# Autodesk Inventor assembly: motormount_new
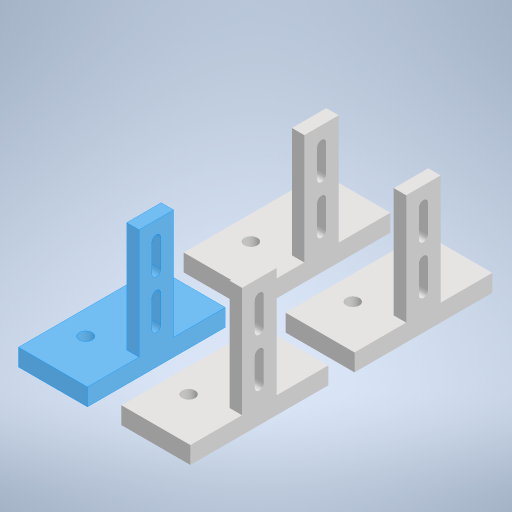
[picture p0: Inventor's stored thumbnail of the model, 512x512]
Saved by Autodesk Inventor 2024 (Build 280153000, 153)
## iProperties
Created: 2023-12-05
Part Number: motormount_new
Document SubType Name: Assembly
Designer: dimademler
Author: dimademler
## Documents named in this file (2)
- \\Mac\Home\Desktop\UCSD\2023-2024\Quarter_1\Physics_124\CAD new motor\motormount_new.iam
- \\Mac\Home\Desktop\UCSD\2023-2024\Quarter_1\Physics_124\CAD new motor\new_motors_adapter.ipt
## Components (4 placed, 1 different names)
1. new_motors_adapter:1 — Flush:1
2. new_motors_adapter:2 — Flush:1, Flush:2
3. new_motors_adapter:3 — Flush:2, Flush:3
4. new_motors_adapter:4 — Flush:3
## Relationships (3: Flush 3)
- Flush:1: new_motors_adapter:1 ↔ new_motors_adapter:2
- Flush:2: new_motors_adapter:2 ↔ new_motors_adapter:3
- Flush:3: new_motors_adapter:3 ↔ new_motors_adapter:4
